# Autodesk Inventor assembly: DeliveryDropArm
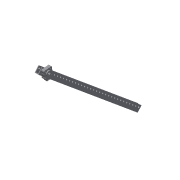
[picture p0: Inventor's stored thumbnail of the model, 180x180]
Saved by Autodesk Inventor 2018 (Build 220112000, 112)
## iProperties
Created: 2018-10-26
Part Number: DeliveryDropArm
Document SubType Name: Assembly
Designer: ball
Author: ball
## Documents named in this file (3)
- C:\FTC\FTC8863CAD\2018Robot\DeliveryDropArm.iam
- C:\FTC\FTC8863CAD\Actobotics\585 parts\585399.ipt
- C:\FTC\FTC8863CAD\Actobotics\545 parts\545619 assembly.ipt
## Components (2 placed, 2 different names)
1. 585399:1 — Mate:1, Mate:2, Mate:3
2. 545619 assembly:2 — Mate:1, Mate:2, Mate:3
## Relationships (3: Mate 3)
- Mate:1: 585399:1 ↔ 545619 assembly:2
- Mate:2: 585399:1 ↔ 545619 assembly:2
- Mate:3: 585399:1 ↔ 545619 assembly:2
